# Autodesk Inventor assembly: tableiam
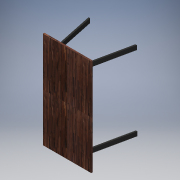
[picture p0: Inventor's stored thumbnail of the model, 180x180]
Saved by Autodesk Inventor 2019 (Build 230136000, 136)
## iProperties
Created: 2019-08-11
Part Number: tableiam
Document SubType Name: Assembly
Designer: Alex
Author: Alex
## Documents named in this file (3)
- P:\Alex\Git\3d_models\dining_table\a-legs\tableiam.iam
- P:\Alex\Git\3d_models\dining_table\a-legs\leg.ipt
- P:\Alex\Git\3d_models\dining_table\a-legs\tabletop.ipt
## Components (3 placed, 2 different names)
1. leg:1 — Mate:2, Flush:1
2. leg:2 — Mate:1, Flush:2
3. tabletop:1 — Mate:1, Mate:2, Flush:1, Flush:2
## Relationships (4: Mate 2, Flush 2)
- Mate:1: leg:2 ↔ tabletop:1
- Mate:2: leg:1 ↔ tabletop:1
- Flush:1 (50 mm): leg:1 ↔ tabletop:1
- Flush:2 (50 mm): leg:2 ↔ tabletop:1
